# Autodesk Inventor assembly: Assembly1
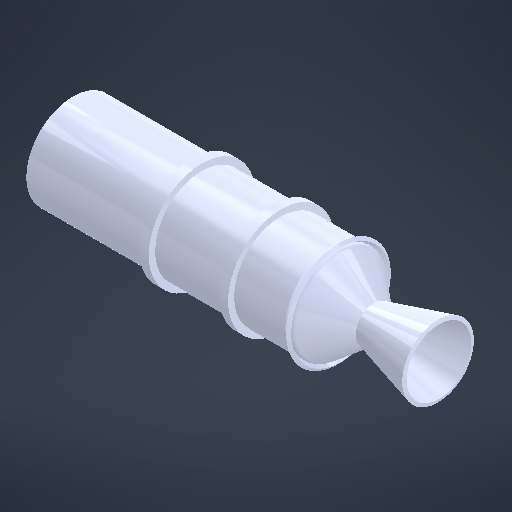
[picture p0: Inventor's stored thumbnail of the model, 512x512]
Saved by Autodesk Inventor 2026.2 (Build 302298000, 298)
## iProperties
Created: 2026-04-04
Part Number: Assembly1
Document SubType Name: Assembly
Designer: athir
Author: athir
## Documents named in this file (4)
- C:\Users\athir\OneDrive\Desktop\Projects\Regeneratively colled liquid rocket engine combustion chamber\Assembly1.iam
- C:\Users\athir\OneDrive\Desktop\Projects\Regeneratively colled liquid rocket engine combustion chamber\part 3\cooling channel system part 2 component1\cooling channel system part 2 component1.ipt
- C:\Users\athir\OneDrive\Desktop\Projects\Regeneratively colled liquid rocket engine combustion chamber\part 3\part 3\part 3.ipt
- C:\Users\athir\OneDrive\Desktop\Projects\Regeneratively colled liquid rocket engine combustion chamber\part 3\Combustion chamber part1\Combustion chamber part1.ipt
## Components (3 placed, 3 different names)
1. cooling channel system part 2 component1:1 — Rotational:1, Rotational:2
2. part 3:1 — Rotational:2
3. Combustion chamber part1:1 — Rotational:1
## Relationships (2: RevoluteJoint 2)
- Rotational:1 [RevoluteJoint] (160.3375 mm): cooling channel system part 2 component1:1 ↔ Combustion chamber part1:1
- Rotational:2 [RevoluteJoint] (-312.7375 mm): cooling channel system part 2 component1:1 ↔ part 3:1
